# Autodesk Inventor assembly: Assembled_Chamber
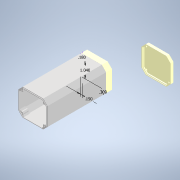
[picture p0: Inventor's stored thumbnail of the model, 180x180]
Saved by Autodesk Inventor 2022 (Build 260153000, 153)
## iProperties
Created: 2021-09-30
Part Number: Assembled_Chamber
Document SubType Name: Assembly
Designer: iss
Author: iss
## Documents named in this file (6)
- C:\Users\r8003\Downloads\Assembled_Chamber.iam
- C:\Users\r8003\Downloads\MicroLab_Center_Shell.ipt
- C:\Users\r8003\Downloads\C329-SPI.ipt
- C:\Users\r8003\Downloads\MicroLab_Rear_Cover.ipt
- C:\Users\r8003\Downloads\MicroLab_Front_Cover.ipt
- C:\Users\r8003\Downloads\MicroLab_PCB_002.ipt
## Components (5 placed, 5 different names)
1. MicroLab_Center_Shell:1 — Flush:2, Mate:5, Mate:6, Mate:13, Mate:14, Mate:21, Angle:1, Flush:5
2. C329-SPI:1 — Mate:16, Mate:17, Mate:18, Flush:6, Flush:7, Flush:9
3. MicroLab_Rear_Cover:1 — Mate:1, Flush:1, Mate:5, Mate:6, Mate:11, Mate:12, Mate:15, Flush:12, Flush:13, Flush:15, Flush:16
4. MicroLab_Front_Cover:1
5. MicroLab_PCB_002:1 — Mate:1, Flush:3, Mate:11, Mate:12, Flush:4, Mate:16, Mate:17, Flush:8
## Relationships (28: Mate 13, Flush 13, Angle 1, Symmetry 1)
- Mate:1: MicroLab_Rear_Cover:1 ↔ MicroLab_PCB_002:1
- Flush:1: MicroLab_Rear_Cover:1
- Flush:2: MicroLab_Center_Shell:1
- Mate:4
- Mate:5: MicroLab_Center_Shell:1 ↔ MicroLab_Rear_Cover:1
- Mate:6: MicroLab_Center_Shell:1 ↔ MicroLab_Rear_Cover:1
- Flush:3 (-17.018 mm): MicroLab_PCB_002:1
- Mate:11: MicroLab_Rear_Cover:1 ↔ MicroLab_PCB_002:1
- Mate:12: MicroLab_Rear_Cover:1 ↔ MicroLab_PCB_002:1
- Mate:13: MicroLab_Center_Shell:1
- Mate:14: MicroLab_Center_Shell:1
- Mate:15: MicroLab_Rear_Cover:1
- Flush:4 (-17.018 mm): MicroLab_PCB_002:1
- Mate:16 (3.429 mm): C329-SPI:1 ↔ MicroLab_PCB_002:1
- Mate:17: C329-SPI:1 ↔ MicroLab_PCB_002:1
- Mate:18: C329-SPI:1
- Mate:21: MicroLab_Center_Shell:1
- Angle:1 (0 deg): MicroLab_Center_Shell:1
- Flush:5: MicroLab_Center_Shell:1
- Flush:6 (4 mm): C329-SPI:1
- Flush:7: C329-SPI:1
- Flush:8 (4 mm): MicroLab_PCB_002:1
- Flush:9: C329-SPI:1
- Flush:12: MicroLab_Rear_Cover:1
- Flush:13: MicroLab_Rear_Cover:1
- Flush:15: MicroLab_Rear_Cover:1
- Flush:16: MicroLab_Rear_Cover:1
- Symmetry:1
